# Autodesk Inventor assembly: RAM-201U-B
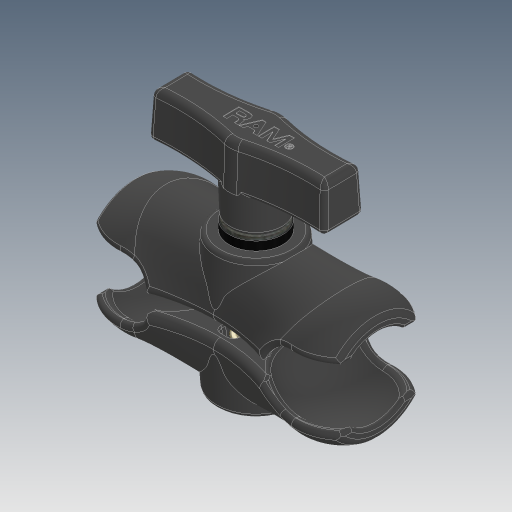
[picture p0: Inventor's stored thumbnail of the model, 512x512]
Saved by Autodesk Inventor 2023.1 (Build 271208000, 208)
## iProperties
Created: 2023-01-30
Part Number: RAM-201U-B
Document SubType Name: Assembly
Designer: Cominelli Nicolas
Mass: 204.972 g
Surface Area: 335.254 cm^2
Volume: 76.9557 cm^3
Density: 2.6635 g/cm^3
Trattamento: -
Author: Cominelli Nicolas
## Documents named in this file (7)
- C:\Users\cominelli.nicolas\Desktop\RAM-201U-B\RAM-201U-B.iam
- C:\Users\cominelli.nicolas\Desktop\RAM-201U-B\Body (RAM-201U-B).ipt
- C:\Users\cominelli.nicolas\Desktop\RAM-201U-B\Bolt (RAM-201U-B).ipt
- C:\Users\cominelli.nicolas\Desktop\RAM-201U-B\Knob (RAM-201U-B).ipt
- C:\Users\cominelli.nicolas\Desktop\RAM-201U-B\Metal Washer (RAM-201U-B).ipt
- C:\Users\cominelli.nicolas\Desktop\RAM-201U-B\Plastic Washer (RAM-201U-B).ipt
- C:\Users\cominelli.nicolas\Desktop\RAM-201U-B\Spring (RAM-201U-B).ipt
## Components (7 placed, 6 different names)
1. Body (RAM-201U-B):1 — Allineato:1, Coincidente:1, Coincidente:2, Inserimento:1, Allineato:2, Coincidente:7
2. Body (RAM-201U-B):2 — Coincidente:5, Coincidente:6, Coincidente:7, Coincidente:9
3. Bolt (RAM-201U-B):1 — Inserimento:1, Coincidente:3, Coincidente:4, Coincidente:8
4. Knob (RAM-201U-B):1 — Inserimento:3
5. Metal Washer (RAM-201U-B):1 — Inserimento:2, Inserimento:3
6. Plastic Washer (RAM-201U-B):1 — Coincidente:8, Coincidente:9, Inserimento:2
7. Spring (RAM-201U-B):1 — Coincidente:4, Allineato:2
## Relationships (14: Mate 9, Insert 3, Flush 2)
- Allineato:1 [Flush]: Body (RAM-201U-B):1
- Coincidente:1 [Mate]: Body (RAM-201U-B):1
- Coincidente:2 [Mate]: Body (RAM-201U-B):1
- Inserimento:1: Body (RAM-201U-B):1 ↔ Bolt (RAM-201U-B):1
- Coincidente:3 [Mate]: Bolt (RAM-201U-B):1
- Coincidente:4 [Mate]: Bolt (RAM-201U-B):1 ↔ Spring (RAM-201U-B):1
- Allineato:2 [Flush]: Body (RAM-201U-B):1 ↔ Spring (RAM-201U-B):1
- Coincidente:5 [Mate]: Body (RAM-201U-B):2
- Coincidente:6 [Mate]: Body (RAM-201U-B):2
- Coincidente:7 [Mate] (5.588 mm): Body (RAM-201U-B):1 ↔ Body (RAM-201U-B):2
- Coincidente:8 [Mate]: Bolt (RAM-201U-B):1 ↔ Plastic Washer (RAM-201U-B):1
- Coincidente:9 [Mate]: Body (RAM-201U-B):2 ↔ Plastic Washer (RAM-201U-B):1
- Inserimento:2: Metal Washer (RAM-201U-B):1 ↔ Plastic Washer (RAM-201U-B):1
- Inserimento:3: Knob (RAM-201U-B):1 ↔ Metal Washer (RAM-201U-B):1
